# Autodesk Inventor assembly: Araknid-4Wire-FDM-C-Slot-x1
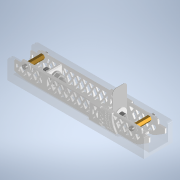
[picture p0: Inventor's stored thumbnail of the model, 180x180]
Saved by Autodesk Inventor 2021 (Build 250183000, 183)
## iProperties
Created: 2020-08-19
Part Number: Araknid-4Wire-FDM-C-Slot-x1
Document SubType Name: Assembly
Designer: lucas
Author: lucas
## Documents named in this file (4)
- C:\Users\lucas\Nextcloud\HackerSpace\HV Home Battery Storage Project\Concepts & Storyboards\18650 4wire Holder\Araknid-4Wire-FDM-C-Slot-x1.iam
- C:\Users\lucas\Nextcloud\HackerSpace\HV Home Battery Storage Project\Concepts & Storyboards\18650 4wire Holder\4Wire-FDM-Slot\FDM-Fixture-x1ipt.ipt
- C:\Users\lucas\Nextcloud\HackerSpace\HV Home Battery Storage Project\Concepts & Storyboards\18650 4wire Holder\4Wire-FDM-Slot\4Wire-FDM-Pivot.iam
- C:\Users\lucas\Nextcloud\HackerSpace\HV Home Battery Storage Project\Concepts & Storyboards\18650 4wire Holder\4Wire-FDM-Slot\4Wire-FDM-Slot.iam
## Components (3 placed, 3 different names)
1. FDM-Fixture-x1ipt:1 — Rotational:1, Rotational:2
2. 4Wire-FDM-Pivot:1 [sub-assembly] — Rotational:1
3. 4Wire-FDM-Slot:1 [sub-assembly] — Rotational:2
## Relationships (2: RevoluteJoint 2)
- Rotational:1 [RevoluteJoint] (0.075 mm): FDM-Fixture-x1ipt:1 ↔ 4Wire-FDM-Pivot:1
- Rotational:2 [RevoluteJoint] (0.075 mm): FDM-Fixture-x1ipt:1 ↔ 4Wire-FDM-Slot:1
